# Autodesk Inventor assembly: X_CarriageR_V2_1
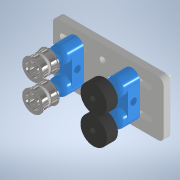
[picture p0: Inventor's stored thumbnail of the model, 180x180]
Saved by Autodesk Inventor 2021 (Build 250183000, 183)
## iProperties
Created: 2021-06-13
Part Number: X_CarriageR_V2_1
Document SubType Name: Assembly
Designer: Jorian Brusind
Author: Jorian Brusind
## Documents named in this file (7)
- C:\Users\Jorian Brusind\Documents\GitHub\HyperRail\Inventor Files\X_CarriageR_V2_1.iam
- C:\Users\Jorian Brusind\Documents\GitHub\HyperRail\Inventor Files\X_Carriage_Plate.ipt
- C:\Users\Jorian Brusind\Documents\GitHub\HyperRail\Inventor Files\4mm_Roller_Spacer_extended.ipt
- C:\Users\Jorian Brusind\Documents\GitHub\HyperRail\Inventor Files\11mm_BearingWheel.ipt
- C:\Users\Jorian Brusind\Documents\GitHub\HyperRail\Inventor Files\Bearing_Spacer.ipt
- C:\Users\Jorian Brusind\Documents\GitHub\HyperRail\Inventor Files\miniature-ball-bearings-metric-series-flanged-1.snapshot.1\F606ZZFlanged\F608 - 8 x 22 x 7.ipt
- C:\Users\Jorian Brusind\Documents\GitHub\PersonalProjects\HyperRail\Inventor Files\miniature-ball-bearings-metric-series-flanged-1.snapshot.1\F606ZZFlanged.ipt
## Components (11 placed, 5 different names)
1. X_Carriage_Plate:1 — Mate:69, Mate:72, Mate:84, Mate:85, Angle:1, Angle:2
2. 4mm_Roller_Spacer_extended:1 — Mate:72, Mate:74, Mate:75, Mate:76, Mate:85, Angle:1
3. 4mm_Roller_Spacer_extended:3 — Mate:69, Mate:84, Angle:2, Mate:95, Mate:96, Mate:97
4. 11mm_BearingWheel:1 — Mate:75, Flush:1, Mate:76
5. 11mm_BearingWheel:2 — Mate:74, Flush:1
6. Bearing_Spacer:1 — Flush:3, Mate:92, Mate:93, Mate:94
7. Bearing_Spacer:2 — Flush:3, Mate:89, Mate:90, Mate:91
8. F608 - 8 x 22 x 7:1 — Mate:92, Mate:94, Mate:96
9. F608 - 8 x 22 x 7:2 — Mate:93
10. F608 - 8 x 22 x 7:3 — Mate:90
11. F608 - 8 x 22 x 7:4 — Mate:89, Mate:91, Mate:95, Mate:97
## Relationships (22: Mate 18, Flush 2, Angle 2)
- Mate:69: X_Carriage_Plate:1 ↔ 4mm_Roller_Spacer_extended:3
- Mate:72: X_Carriage_Plate:1 ↔ 4mm_Roller_Spacer_extended:1
- Mate:74: 4mm_Roller_Spacer_extended:1 ↔ 11mm_BearingWheel:2
- Mate:75: 4mm_Roller_Spacer_extended:1 ↔ 11mm_BearingWheel:1
- Flush:1: 11mm_BearingWheel:1 ↔ 11mm_BearingWheel:2
- Mate:76: 4mm_Roller_Spacer_extended:1 ↔ 11mm_BearingWheel:1
- Mate:84 (-12.5 mm): X_Carriage_Plate:1 ↔ 4mm_Roller_Spacer_extended:3
- Mate:85 (-12.5 mm): X_Carriage_Plate:1 ↔ 4mm_Roller_Spacer_extended:1
- Angle:1 (0 deg): X_Carriage_Plate:1 ↔ 4mm_Roller_Spacer_extended:1
- Angle:2 (0 deg): X_Carriage_Plate:1 ↔ 4mm_Roller_Spacer_extended:3
- Flush:3: Bearing_Spacer:1 ↔ Bearing_Spacer:2
- [Mate]: F608 - 8 x 22 x 7:1 ↔ F608 - 8 x 22 x 7:2
- [Mate]: F608 - 8 x 22 x 7:3 ↔ F608 - 8 x 22 x 7:4
- Mate:89: Bearing_Spacer:2 ↔ F608 - 8 x 22 x 7:4
- Mate:90: Bearing_Spacer:2 ↔ F608 - 8 x 22 x 7:3
- Mate:91: Bearing_Spacer:2 ↔ F608 - 8 x 22 x 7:4
- Mate:92: Bearing_Spacer:1 ↔ F608 - 8 x 22 x 7:1
- Mate:93: Bearing_Spacer:1 ↔ F608 - 8 x 22 x 7:2
- Mate:94: Bearing_Spacer:1 ↔ F608 - 8 x 22 x 7:1
- Mate:95: 4mm_Roller_Spacer_extended:3 ↔ F608 - 8 x 22 x 7:4
- Mate:96: 4mm_Roller_Spacer_extended:3 ↔ F608 - 8 x 22 x 7:1
- Mate:97: 4mm_Roller_Spacer_extended:3 ↔ F608 - 8 x 22 x 7:4
## Named parameters: d136_d94 = 0 mm
